# Autodesk Inventor assembly: OBSN-30-B
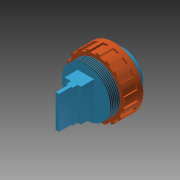
[picture p0: Inventor's stored thumbnail of the model, 180x180]
Saved by Autodesk Inventor 2013 (Build 170138000, 138)
## iProperties
Created: 2012-06-18
Part Number: OBSN-30-B
Document SubType Name: Assembly
Designer: mstine
Author: mstine
## Documents named in this file (3)
- C:\Users\mstine\Desktop\software\Pew-Pew-Stick\assemblies\OBSN-30-B.iam
- C:\Users\mstine\Desktop\software\Pew-Pew-Stick\parts\OBSN-30-B_button.ipt
- C:\Users\mstine\Desktop\software\Pew-Pew-Stick\parts\OBSN-30-B_ring.ipt
## Components (2 placed, 2 different names)
1. OBSN-30-B_button:1 — Mate:1, Mate:2
2. OBSN-30-B_ring:1 — Mate:1, Mate:2
## Relationships (2: Mate 2)
- Mate:1: OBSN-30-B_button:1 ↔ OBSN-30-B_ring:1
- Mate:2: OBSN-30-B_button:1 ↔ OBSN-30-B_ring:1
